# Autodesk Inventor assembly: Enclosure
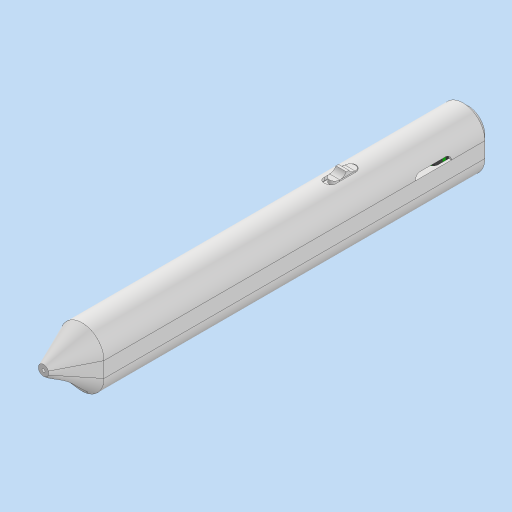
[picture p0: Inventor's stored thumbnail of the model, 512x512]
Saved by Autodesk Inventor 2024 (Build 280153000, 153)
## iProperties
Created: 2025-02-15
Part Number: Enclosure
Document SubType Name: Assembly
Designer: XxPan
Author: XxPan
## Documents named in this file (11)
- C:\Users\XxPan\OneDrive - McMaster University\4OI6\InkSync\case\Enclosure.iam
- C:\Users\XxPan\OneDrive - McMaster University\4OI6\InkSync\case\MCU_PCB.iam
- C:\Users\XxPan\OneDrive - McMaster University\4OI6\InkSync\case\Sensor_PCB.iam
- C:\Users\XxPan\OneDrive - McMaster University\4OI6\InkSync\case\Battery.ipt
- C:\Users\XxPan\OneDrive - McMaster University\4OI6\InkSync\case\Shell.ipt
- C:\Users\XxPan\OneDrive - McMaster University\4OI6\InkSync\case\Power_switch.ipt
- C:\Users\XxPan\OneDrive - McMaster University\4OI6\InkSync\case\Spring_pin.ipt
- C:\Users\XxPan\OneDrive - McMaster University\4OI6\InkSync\case\Shell_body_top.ipt
- C:\Users\XxPan\OneDrive - McMaster University\4OI6\InkSync\case\Sliding_switch.ipt
- C:\Users\XxPan\OneDrive - McMaster University\4OI6\InkSync\case\OMGUSB.ipt
- C:\Users\XxPan\OneDrive - McMaster University\4OI6\InkSync\case\Display_stand\Display_stand.ipt
## Components (10 placed, 10 different names)
1. MCU_PCB:1 [sub-assembly]
2. Sensor_PCB:1 [sub-assembly] — Flush:5, Flush:6, Flush:7, Flush:8, Flush:11
3. Battery:1 — Angle:1, Insert:2
4. Shell:1 — Flush:11, Insert:1, Angle:1, Insert:2, Insert:3, Mate:7, Insert:4, Angle:2, Insert:5
5. Power_switch:1 — Flush:15, Flush:14, Flush:16, Mate:10
6. Spring_pin:1 — Insert:1
7. Shell_body_top:1 — Insert:3, Mate:7, Mate:9
8. Sliding_switch:1 — Mate:8, Mate:9, Mate:10
9. OMGUSB:1 — Insert:4, Angle:2
10. Display_stand:1 — Insert:5
## Relationships (19: Flush 8, Insert 5, Mate 4, Angle 2)
- Flush:5: Sensor_PCB:1
- Flush:6: Sensor_PCB:1
- Flush:7: Sensor_PCB:1
- Flush:8: Sensor_PCB:1
- Flush:11 (12 mm): Sensor_PCB:1 ↔ Shell:1
- Flush:15: Power_switch:1
- Flush:14: Power_switch:1
- Flush:16 (-95 mm): Power_switch:1
- Insert:1: Shell:1 ↔ Spring_pin:1
- Angle:1 (180 deg): Battery:1 ↔ Shell:1
- Insert:2 (-25 mm): Battery:1 ↔ Shell:1
- Insert:3: Shell:1 ↔ Shell_body_top:1
- Mate:7: Shell:1 ↔ Shell_body_top:1
- Mate:8: Sliding_switch:1
- Mate:9: Shell_body_top:1 ↔ Sliding_switch:1
- Mate:10 (0.2 mm): Power_switch:1 ↔ Sliding_switch:1
- Insert:4: Shell:1 ↔ OMGUSB:1
- Angle:2 (180 deg): Shell:1 ↔ OMGUSB:1
- Insert:5 (-60 mm): Shell:1 ↔ Display_stand:1
